# Autodesk Inventor assembly: szafka
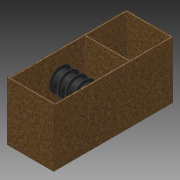
[picture p0: Inventor's stored thumbnail of the model, 180x180]
Saved by Autodesk Inventor 2013 (Build 170138000, 138)
## iProperties
Created: 2014-04-26
Part Number: szafka
Document SubType Name: Assembly
Designer: Masta
Author: Masta
## Documents named in this file (7)
- D:\prusa i3\szafka\szafka.iam
- D:\prusa i3\szafka\bok.ipt
- D:\prusa i3\szafka\tyl.ipt
- D:\prusa i3\szafka\podstawa.ipt
- D:\prusa i3\szafka\polka.ipt
- D:\prusa i3\szafka\rolka_filamentu.ipt
- D:\prusa i3\szafka\gora.ipt
## Components (11 placed, 6 different names)
1. bok:1 — Flush:2, Flush:5, Mate:5, Flush:7, Mate:10, Flush:9
2. bok:2 — Flush:8, Mate:6, Mate:7
3. tyl:1 — Mate:1, Flush:2, Mate:4, Flush:6, Mate:5, Flush:7, Flush:8, Mate:6, Mate:9, Mate:11, Flush:10
4. podstawa:1 — Mate:4, Flush:5, Flush:6, Mate:7
5. polka:1 — Mate:9, Mate:10
6. rolka_filamentu:1 — Insert:1, Insert:2
7. rolka_filamentu:2 — Insert:1, Insert:3
8. rolka_filamentu:3 — Insert:3
9. rolka_filamentu:4 — Insert:2, Insert:4
10. gora:1 — Mate:11, Flush:9, Flush:10
11. rolka_filamentu:5 — Insert:4
## Relationships (19: Mate 8, Flush 7, Insert 4)
- Mate:1: tyl:1
- Flush:2: bok:1 ↔ tyl:1
- Mate:4: tyl:1 ↔ podstawa:1
- Flush:5: bok:1 ↔ podstawa:1
- Flush:6: tyl:1 ↔ podstawa:1
- Mate:5: bok:1 ↔ tyl:1
- Flush:7: bok:1 ↔ tyl:1
- Flush:8: bok:2 ↔ tyl:1
- Mate:6: bok:2 ↔ tyl:1
- Mate:7: bok:2 ↔ podstawa:1
- Mate:9: tyl:1 ↔ polka:1
- Mate:10: bok:1 ↔ polka:1
- Mate:11: tyl:1 ↔ gora:1
- Flush:9: bok:1 ↔ gora:1
- Flush:10: tyl:1 ↔ gora:1
- Insert:1: rolka_filamentu:1 ↔ rolka_filamentu:2
- Insert:2: rolka_filamentu:1 ↔ rolka_filamentu:4
- Insert:3: rolka_filamentu:2 ↔ rolka_filamentu:3
- Insert:4: rolka_filamentu:4 ↔ rolka_filamentu:5
